# Autodesk Inventor assembly: Assembly1
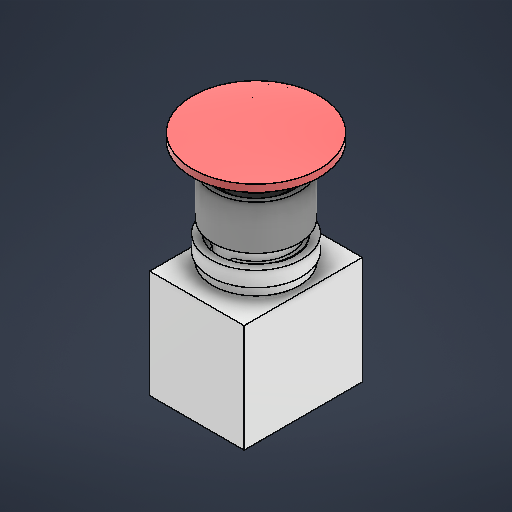
[picture p0: Inventor's stored thumbnail of the model, 512x512]
Saved by Autodesk Inventor 2026 (Build 300175050, 175E)
## iProperties
Created: 2025-06-28
Part Number: Assembly1
Document SubType Name: Assembly
Designer: Joshua Eah
Author: Joshua Eah
## Documents named in this file (6)
- C:\Users\Joshua Eah\Documents\GitHub\Voron-0\CAD\Master Assembly\Extras\E-Stop\Assembly1.iam
- C:\Users\Joshua Eah\Documents\GitHub\Voron-0\CAD\Master Assembly\Extras\E-Stop\Body.ipt
- C:\Users\Joshua Eah\Documents\GitHub\Voron-0\CAD\Master Assembly\Extras\E-Stop\Bottom Nut.ipt
- C:\Users\Joshua Eah\Documents\GitHub\Voron-0\CAD\Master Assembly\Extras\E-Stop\Top Nut.ipt
- C:\Users\Joshua Eah\Documents\GitHub\Voron-0\CAD\Master Assembly\Extras\E-Stop\Plunger.ipt
- C:\Users\Joshua Eah\Documents\GitHub\Voron-0\CAD\Master Assembly\Extras\E-Stop\E-Stop Button.ipt
## Components (5 placed, 5 different names)
1. Body:1 — Insert:1, Insert:2, Mate:1
2. Bottom Nut:1 — Insert:1
3. Top Nut:1 — Insert:2, Mate:2
4. Plunger:1 — Mate:1, Mate:2, Mate:3, Mate:4
5. E-Stop Button:1 — Mate:3, Mate:4
## Relationships (6: Mate 4, Insert 2)
- Insert:1: Body:1 ↔ Bottom Nut:1
- Insert:2: Body:1 ↔ Top Nut:1
- Mate:1: Body:1 ↔ Plunger:1
- Mate:2: Top Nut:1 ↔ Plunger:1
- Mate:3: Plunger:1 ↔ E-Stop Button:1
- Mate:4: Plunger:1 ↔ E-Stop Button:1
